# Autodesk Inventor assembly: Shift Knob Assembly
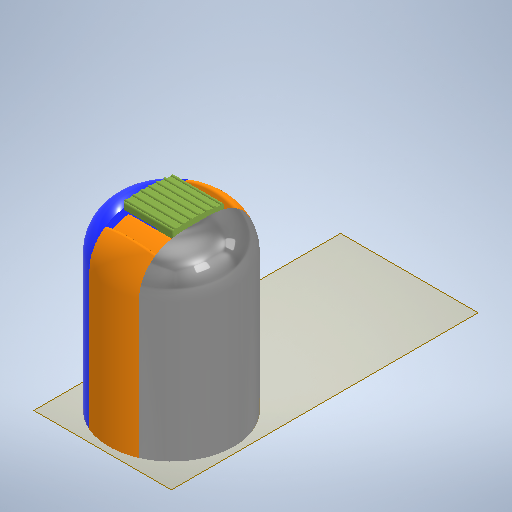
[picture p0: Inventor's stored thumbnail of the model, 512x512]
Saved by Autodesk Inventor 2025.2 (Build 292293000, 293)
## iProperties
Created: 2025-02-16
Part Number: Shift Knob Assembly
Document SubType Name: Assembly
Designer: eason
Author: eason
## Documents named in this file (5)
- C:\Users\eason\Desktop\Code\Unojoy-Simulator-Rig\CAD\Shift Knob\Shift Knob Assembly.iam
- C:\Users\eason\Desktop\Code\Unojoy-Simulator-Rig\CAD\Shift Knob\Joystick.ipt
- C:\Users\eason\Desktop\Code\Unojoy-Simulator-Rig\CAD\Shift Knob\Middle.ipt
- C:\Users\eason\Desktop\Code\Unojoy-Simulator-Rig\CAD\Shift Knob\Pot Side.ipt
- C:\Users\eason\Desktop\Code\Unojoy-Simulator-Rig\CAD\Shift Knob\Switch Side.ipt
## Components (4 placed, 4 different names)
1. Middle:1 — Mate:1, Mate:2, Flush:1, Insert:1, Cylindrical:1, Insert:2
2. Pot Side:1 — Insert:1, Insert:2, Insert:3, Insert:4
3. Joystick:1 — Flush:1, Cylindrical:1
4. Switch Side:1 — Insert:3, Insert:4
## Relationships (8: Insert 4, Mate 2, Flush 1, CylindricalJoint 1)
- Mate:1: Middle:1
- Mate:2: Middle:1
- Flush:1: Middle:1 ↔ Joystick:1
- Insert:1: Middle:1 ↔ Pot Side:1
- Cylindrical:1: Middle:1 ↔ Joystick:1
- Insert:2: Middle:1 ↔ Pot Side:1
- Insert:3: Pot Side:1 ↔ Switch Side:1
- Insert:4: Pot Side:1 ↔ Switch Side:1
